# Autodesk Inventor assembly: ClimbBase-1111-2020
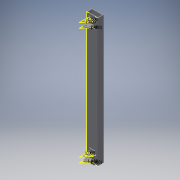
[picture p0: Inventor's stored thumbnail of the model, 180x180]
Saved by Autodesk Inventor 2018 (Build 220112000, 112)
## iProperties
Created: 2020-02-07
Part Number: ClimbBase-1111-2020
Document SubType Name: Assembly
Designer: JMHal
Author: JMHal
## Documents named in this file (4)
- E:\PHRC CADD\2020 Infinite Recharge\Lift\Assemblies\ClimbBase-1111-2020.iam
- E:\PHRC CADD\2020 Infinite Recharge\Lift\Parts\LiftBase-1111-2020.ipt
- E:\PHRC CADD\Resources\Pneumatic Resources\LeftPinAtttachments-1111-2019.ipt
- E:\PHRC CADD\Resources\Pneumatic Resources\LeftPinAtttachments-1111-2019_MIR.ipt
## Components (5 placed, 3 different names)
1. LiftBase-1111-2020:1 — Mate:1, Mate:2, Flush:1, Mate:6, Mate:7, Flush:4, Flush:5, Flush:6
2. LeftPinAtttachments-1111-2019:1 — Mate:1, Mate:5, Flush:2, Flush:6
3. LeftPinAtttachments-1111-2019_MIR:1 — Mate:2, Mate:5, Flush:1, Flush:2
4. LeftPinAtttachments-1111-2019_MIR:2 — Mate:6, Flush:3, Mate:8, Flush:5
5. LeftPinAtttachments-1111-2019:2 — Mate:7, Flush:3, Flush:4, Mate:8
## Relationships (12: Mate 6, Flush 6)
- Mate:1: LiftBase-1111-2020:1 ↔ LeftPinAtttachments-1111-2019:1
- Mate:2: LiftBase-1111-2020:1 ↔ LeftPinAtttachments-1111-2019_MIR:1
- Mate:5 (15.748 mm): LeftPinAtttachments-1111-2019:1 ↔ LeftPinAtttachments-1111-2019_MIR:1
- Flush:1 (11.1125 mm): LiftBase-1111-2020:1 ↔ LeftPinAtttachments-1111-2019_MIR:1
- Flush:2: LeftPinAtttachments-1111-2019:1 ↔ LeftPinAtttachments-1111-2019_MIR:1
- Mate:6: LiftBase-1111-2020:1 ↔ LeftPinAtttachments-1111-2019_MIR:2
- Mate:7: LiftBase-1111-2020:1 ↔ LeftPinAtttachments-1111-2019:2
- Flush:3: LeftPinAtttachments-1111-2019_MIR:2 ↔ LeftPinAtttachments-1111-2019:2
- Flush:4 (11.1125 mm): LiftBase-1111-2020:1 ↔ LeftPinAtttachments-1111-2019:2
- Mate:8 (15.748 mm): LeftPinAtttachments-1111-2019_MIR:2 ↔ LeftPinAtttachments-1111-2019:2
- Flush:5 (2.794 mm): LiftBase-1111-2020:1 ↔ LeftPinAtttachments-1111-2019_MIR:2
- Flush:6 (-2.794 mm): LiftBase-1111-2020:1 ↔ LeftPinAtttachments-1111-2019:1
